# Autodesk Inventor assembly: BatteryPack
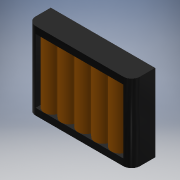
[picture p0: Inventor's stored thumbnail of the model, 180x180]
Saved by Autodesk Inventor 2018 (Build 220112000, 112)
## iProperties
Created: 2018-01-13
Part Number: BatteryPack
Document SubType Name: Assembly
Designer: Kyle-HP
Author: Kyle-HP
## Documents named in this file (3)
- C:\Users\Kyle-HP\Documents\Hackathon-2018\Inventor\Robot\BatteryPack.iam
- C:\Users\Kyle-HP\Documents\Hackathon-2018\Inventor\Robot\BatteryHolder.ipt
- C:\Users\Kyle-HP\Documents\Hackathon-2018\Inventor\Robot\Battery.ipt
## Components (6 placed, 2 different names)
1. BatteryHolder:1 — Mate:1, Mate:2, Tangent:1, Mate:3, Tangent:2, Mate:4, Mate:5, Tangent:3, Mate:6, Mate:7, Tangent:4, Mate:8, Mate:9, Tangent:5, Mate:10
2. Battery:1 — Mate:1, Mate:2, Tangent:1
3. Battery:2 — Mate:3, Tangent:2, Mate:4
4. Battery:3 — Mate:5, Tangent:3, Mate:6
5. Battery:4 — Mate:7, Tangent:4, Mate:8
6. Battery:5 — Mate:9, Tangent:5, Mate:10
## Relationships (15: Mate 10, Tangent 5)
- Mate:1: BatteryHolder:1 ↔ Battery:1
- Mate:2 (6.35 mm): BatteryHolder:1 ↔ Battery:1
- Tangent:1: BatteryHolder:1 ↔ Battery:1
- Mate:3: BatteryHolder:1 ↔ Battery:2
- Tangent:2: BatteryHolder:1 ↔ Battery:2
- Mate:4 (19.05 mm): BatteryHolder:1 ↔ Battery:2
- Mate:5: BatteryHolder:1 ↔ Battery:3
- Tangent:3: BatteryHolder:1 ↔ Battery:3
- Mate:6 (31.75 mm): BatteryHolder:1 ↔ Battery:3
- Mate:7: BatteryHolder:1 ↔ Battery:4
- Tangent:4: BatteryHolder:1 ↔ Battery:4
- Mate:8 (44.45 mm): BatteryHolder:1 ↔ Battery:4
- Mate:9: BatteryHolder:1 ↔ Battery:5
- Tangent:5: BatteryHolder:1 ↔ Battery:5
- Mate:10 (57.15 mm): BatteryHolder:1 ↔ Battery:5
